# Autodesk Inventor assembly: Cryostat
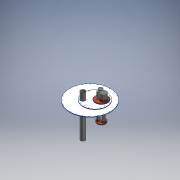
[picture p0: Inventor's stored thumbnail of the model, 180x180]
Saved by Autodesk Inventor 2018 (Build 220112000, 112)
## iProperties
Created: 2018-10-10
Part Number: Cryostat
Document SubType Name: Assembly
Designer: Admin
Author: Admin
## Documents named in this file (8)
- C:\Users\freyja\Documents\Cryorefrigerator\CAD\Cryostat.iam
- C:\Users\freyja\Documents\Cryorefrigerator\CAD\External Models\CH40415 24JUL14 C.ipt
- C:\Users\freyja\Documents\Cryorefrigerator\CAD\vacuum jacket long.ipt
- C:\Users\freyja\Documents\Cryorefrigerator\CAD\vacuum jacket.ipt
- C:\Users\freyja\Documents\Cryorefrigerator\CAD\Top Plate V2.2.ipt
- C:\Users\freyja\Documents\Cryorefrigerator\CAD\still pipe standin.ipt
- C:\Users\freyja\Documents\Cryorefrigerator\CAD\55K stage.ipt
- C:\Users\freyja\Documents\Cryorefrigerator\CAD\mini 55K stage.ipt
## Components (7 placed, 7 different names)
1. Top Plate V2.2:1 — Mate:16, Mate:18, Mate:19, Mate:20, Mate:21, Mate:26, Mate:47
2. CH40415 24JUL14 C:1 — Mate:16, Mate:18, Mate:26, Mate:49, Flush:1
3. vacuum jacket long:1 — Mate:7, Mate:8, Mate:9
4. vacuum jacket:1 — Mate:7, Mate:8, Mate:9, Mate:19, Mate:20, Mate:21
5. still pipe standin:1 — Mate:47, Mate:48
6. 55K stage:1 — Mate:51, Mate:52, Mate:53
7. mini 55K stage:1 — Mate:48, Mate:49, Flush:1, Mate:51, Mate:52, Mate:53
## Relationships (16: Mate 15, Flush 1)
- Mate:7: vacuum jacket long:1 ↔ vacuum jacket:1
- Mate:8: vacuum jacket long:1 ↔ vacuum jacket:1
- Mate:9: vacuum jacket long:1 ↔ vacuum jacket:1
- Mate:16: Top Plate V2.2:1 ↔ CH40415 24JUL14 C:1
- Mate:18: Top Plate V2.2:1 ↔ CH40415 24JUL14 C:1
- Mate:19: Top Plate V2.2:1 ↔ vacuum jacket:1
- Mate:20: Top Plate V2.2:1 ↔ vacuum jacket:1
- Mate:21: Top Plate V2.2:1 ↔ vacuum jacket:1
- Mate:26: Top Plate V2.2:1 ↔ CH40415 24JUL14 C:1
- Mate:47: Top Plate V2.2:1 ↔ still pipe standin:1
- Mate:48: still pipe standin:1 ↔ mini 55K stage:1
- Mate:49: CH40415 24JUL14 C:1 ↔ mini 55K stage:1
- Flush:1: CH40415 24JUL14 C:1 ↔ mini 55K stage:1
- Mate:51: 55K stage:1 ↔ mini 55K stage:1
- Mate:52: 55K stage:1 ↔ mini 55K stage:1
- Mate:53: 55K stage:1 ↔ mini 55K stage:1
